# Autodesk Inventor assembly: Sheathing_For_Side
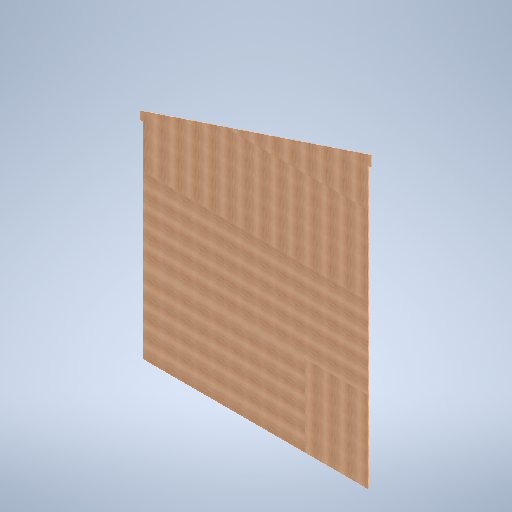
[picture p0: Inventor's stored thumbnail of the model, 512x512]
Saved by Autodesk Inventor 2025 (Build 290162010, 162A)
## iProperties
Created: 2024-10-03
Part Number: Sheathing_For_Side
Document SubType Name: Assembly
Designer: Tom
Author: Tom
## Documents named in this file (8)
- C:\Users\Tom\Documents\Inventor\Mobility\Additional_Building\Sheathing_For_Side.iam
- C:\Users\Tom\Documents\Inventor\Mobility\Additional_Building\OSB_For_Walls_With_Dimensions_48_x_96_Inches.ipt
- C:\Users\Tom\Documents\Inventor\Mobility\Additional_Building\OSB_For_Walls_With_Dimensions_48_x_48_Inches.ipt
- C:\Users\Tom\Documents\Inventor\Mobility\Additional_Building\OSB_For_Walls_With_Dimensions_48_x_85_Inches.ipt
- C:\Users\Tom\Documents\Inventor\Mobility\Additional_Building\OSB_For_Side_And_Back.ipt
- C:\Users\Tom\Documents\Inventor\Mobility\Additional_Building\OSB_For_Walls_With_Dimensions_38.375_x_46.63743616_Inches.ipt
- C:\Users\Tom\Documents\Inventor\Mobility\Additional_Building\OSB_For_Side_And_Top.ipt
- C:\Users\Tom\Documents\Inventor\Mobility\Additional_Building\OSB_For_Walls_With_Dimensions_37_x_48_Inches.ipt
## Components (7 placed, 7 different names)
1. OSB_For_Walls_With_Dimensions_48_x_96_Inches:1 — Mate:1, Mate:2, Mate:3, Mate:5, Flush:3, Flush:4, Flush:11, Flush:12, Mate:12, Mate:13, Flush:20, Flush:21, Flush:22, Flush:23, Flush:25, Flush:26
2. OSB_For_Walls_With_Dimensions_48_x_48_Inches:1 — Mate:5, Flush:3, Flush:4, Mate:7, Mate:8, Flush:5, Flush:6, Flush:11, Flush:15, Flush:16, Flush:22
3. OSB_For_Walls_With_Dimensions_48_x_85_Inches:1 — Mate:7, Flush:12, Flush:15, Mate:11, Mate:13, Flush:21
4. OSB_For_Side_And_Back:1 — Mate:8, Flush:5, Flush:6, Flush:16, Flush:18, Flush:23, Mate:14, Mate:16
5. OSB_For_Side_And_Top:1 — Flush:18, Flush:25, Mate:15, Mate:16, Flush:27
6. OSB_For_Walls_With_Dimensions_37_x_48_Inches:1 — Mate:11, Mate:12, Flush:20
7. OSB_For_Walls_With_Dimensions_38.375_x_46.63743616_Inches:1 — Mate:14, Mate:15, Flush:26, Flush:27
## Relationships (28: Flush 16, Mate 12)
- Mate:1: OSB_For_Walls_With_Dimensions_48_x_96_Inches:1
- Mate:2: OSB_For_Walls_With_Dimensions_48_x_96_Inches:1
- Mate:3: OSB_For_Walls_With_Dimensions_48_x_96_Inches:1
- Mate:5: OSB_For_Walls_With_Dimensions_48_x_96_Inches:1 ↔ OSB_For_Walls_With_Dimensions_48_x_48_Inches:1
- Flush:3: OSB_For_Walls_With_Dimensions_48_x_96_Inches:1 ↔ OSB_For_Walls_With_Dimensions_48_x_48_Inches:1
- Flush:4: OSB_For_Walls_With_Dimensions_48_x_96_Inches:1 ↔ OSB_For_Walls_With_Dimensions_48_x_48_Inches:1
- Mate:7: OSB_For_Walls_With_Dimensions_48_x_48_Inches:1 ↔ OSB_For_Walls_With_Dimensions_48_x_85_Inches:1
- Mate:8: OSB_For_Walls_With_Dimensions_48_x_48_Inches:1 ↔ OSB_For_Side_And_Back:1
- Flush:5: OSB_For_Walls_With_Dimensions_48_x_48_Inches:1 ↔ OSB_For_Side_And_Back:1
- Flush:6: OSB_For_Walls_With_Dimensions_48_x_48_Inches:1 ↔ OSB_For_Side_And_Back:1
- Flush:11: OSB_For_Walls_With_Dimensions_48_x_96_Inches:1 ↔ OSB_For_Walls_With_Dimensions_48_x_48_Inches:1
- Flush:12: OSB_For_Walls_With_Dimensions_48_x_96_Inches:1 ↔ OSB_For_Walls_With_Dimensions_48_x_85_Inches:1
- Flush:15: OSB_For_Walls_With_Dimensions_48_x_48_Inches:1 ↔ OSB_For_Walls_With_Dimensions_48_x_85_Inches:1
- Flush:16: OSB_For_Walls_With_Dimensions_48_x_48_Inches:1 ↔ OSB_For_Side_And_Back:1
- Flush:18: OSB_For_Side_And_Back:1 ↔ OSB_For_Side_And_Top:1
- Mate:11: OSB_For_Walls_With_Dimensions_48_x_85_Inches:1 ↔ OSB_For_Walls_With_Dimensions_37_x_48_Inches:1
- Mate:12: OSB_For_Walls_With_Dimensions_48_x_96_Inches:1 ↔ OSB_For_Walls_With_Dimensions_37_x_48_Inches:1
- Mate:13: OSB_For_Walls_With_Dimensions_48_x_96_Inches:1 ↔ OSB_For_Walls_With_Dimensions_48_x_85_Inches:1
- Flush:20: OSB_For_Walls_With_Dimensions_48_x_96_Inches:1 ↔ OSB_For_Walls_With_Dimensions_37_x_48_Inches:1
- Flush:21: OSB_For_Walls_With_Dimensions_48_x_96_Inches:1 ↔ OSB_For_Walls_With_Dimensions_48_x_85_Inches:1
- Flush:22: OSB_For_Walls_With_Dimensions_48_x_96_Inches:1 ↔ OSB_For_Walls_With_Dimensions_48_x_48_Inches:1
- Flush:23: OSB_For_Walls_With_Dimensions_48_x_96_Inches:1 ↔ OSB_For_Side_And_Back:1
- Flush:25: OSB_For_Walls_With_Dimensions_48_x_96_Inches:1 ↔ OSB_For_Side_And_Top:1
- Mate:14: OSB_For_Side_And_Back:1 ↔ OSB_For_Walls_With_Dimensions_38.375_x_46.63743616_Inches:1
- Mate:15: OSB_For_Side_And_Top:1 ↔ OSB_For_Walls_With_Dimensions_38.375_x_46.63743616_Inches:1
- Flush:26: OSB_For_Walls_With_Dimensions_48_x_96_Inches:1 ↔ OSB_For_Walls_With_Dimensions_38.375_x_46.63743616_Inches:1
- Mate:16: OSB_For_Side_And_Back:1 ↔ OSB_For_Side_And_Top:1
- Flush:27: OSB_For_Side_And_Top:1 ↔ OSB_For_Walls_With_Dimensions_38.375_x_46.63743616_Inches:1
